# Autodesk Inventor assembly: inner
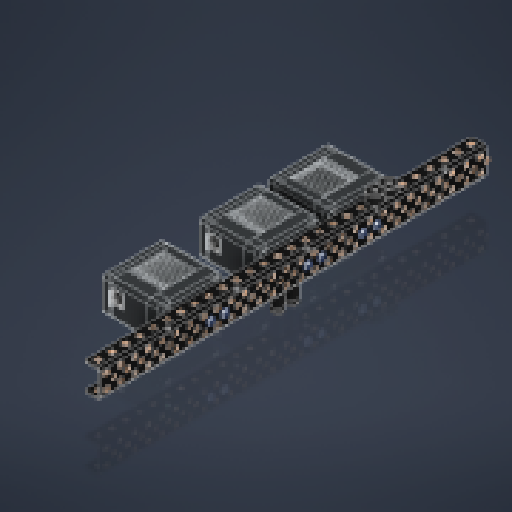
[picture p0: Inventor's stored thumbnail of the model, 512x512]
Saved by Autodesk Inventor 2024 (Build 280153000, 153)
## iProperties
Created: 2024-02-11
Part Number: inner
Document SubType Name: Assembly
Designer: Averey Ku
Author: Averey Ku
## Documents named in this file (15)
- D:\vex_robotics\hardware\cad\vroomba_v0.1\chassis\drivebay\inner.iam
- D:\vex_robotics\hardware\cad\VEX-CAD-Inventor-1.41\Structure\C Channel\Aluminum 1x2x1\Alu C 1x2x1x28.ipt
- D:\vex_robotics\hardware\cad\VEX-CAD-Inventor-1.41\Electronics\Motors with Screws\SteelM-StarS.iam
- D:\vex_robotics\hardware\cad\VEX-CAD-Inventor-1.41\Electronics\Motors with Screws.iam
- D:\vex_robotics\hardware\cad\VEX-CAD-Inventor-1.41\Motion\Shaft LS\Bearing Flat Low Profile.ipt
- D:\vex_robotics\hardware\cad\VEX-CAD-Inventor-1.41\Motion\Spacers\Spacer Nylon .500 OD\NSpacer Black .500 OD x .250.ipt
- D:\vex_robotics\hardware\cad\VEX-CAD-Inventor-1.41\Motion\Spacers\Spacer Nylon .500 OD.ipt
- D:\vex_robotics\hardware\cad\VEX-CAD-Inventor-1.41\Motion\Spacers\Washer Delrin\DWasher .500 OD x .062500.ipt
- D:\vex_robotics\hardware\cad\VEX-CAD-Inventor-1.41\Structure\Hardware\Nut Low Profile.ipt
- D:\vex_robotics\hardware\cad\VEX-CAD-Inventor-1.41\Structure\1-Post Standoff Retainer.ipt
- D:\vex_robotics\hardware\cad\VEX-CAD-Inventor-1.41\Motion\Spacers\Spacer Nylon .375 OD\NSpacer .375 OD x .500.ipt
- D:\vex_robotics\hardware\cad\VEX-CAD-Inventor-1.41\Motion\Spacers\Spacer Nylon .375 OD.ipt
- D:\vex_robotics\hardware\cad\VEX-CAD-Inventor-1.41\Motion\Spacers\Spacer Nylon .375 OD\NSpacer .375 OD x .125.ipt
- D:\vex_robotics\hardware\cad\VEX-CAD-Inventor-1.41\Motion\Spacers\Washer Steel\SWasher .375 OD x .062500.ipt
- D:\vex_robotics\hardware\cad\VEX-CAD-Inventor-1.41\Motion\Spacers\Washer Steel.ipt
## Components (22 placed, 10 different names)
1. Alu C 1x2x1x28:1 — Insert:1, Mate:1, Insert:2, Mate:2, Insert:3, Mate:3, Insert:4, Mate:4, Insert:5, Mate:5, Insert:6, Mate:6, Insert:7, Mate:7, Insert:10, Insert:11, Insert:14, Insert:15, Mate:8, Mate:9, Insert:20, Insert:21
2. SteelM-StarS:1 [sub-assembly] — Insert:3, Mate:3
3. SteelM-StarS:2 [sub-assembly] — Insert:2, Mate:2
4. SteelM-StarS:3 [sub-assembly] — Insert:1, Mate:1
5. Bearing Flat Low Profile:1 — Insert:4, Mate:4
6. Bearing Flat Low Profile:2 — Insert:5, Mate:5
7. Bearing Flat Low Profile:3 — Insert:6, Mate:6
8. Bearing Flat Low Profile:4 — Insert:7, Mate:7
9. NSpacer Black .500 OD x .250:1 — Insert:11
10. DWasher .500 OD x .062500:1
11. NSpacer Black .500 OD x .250:2 — Insert:10
12. DWasher .500 OD x .062500:2
13. Nut Low Profile:1
14. 1-Post Standoff Retainer:1 — Insert:15, Mate:8
15. Nut Low Profile:2
16. 1-Post Standoff Retainer:2 — Insert:14, Mate:9
17. NSpacer .375 OD x .500:1 — Insert:20
18. NSpacer .375 OD x .125:2
19. SWasher .375 OD x .062500:1
20. NSpacer .375 OD x .500:3 — Insert:21
21. NSpacer .375 OD x .125:4
22. SWasher .375 OD x .062500:2
## Relationships (30: Insert 21, Mate 9)
- Insert:1: Alu C 1x2x1x28:1 ↔ SteelM-StarS:3
- Mate:1: Alu C 1x2x1x28:1 ↔ SteelM-StarS:3
- Insert:2: Alu C 1x2x1x28:1 ↔ SteelM-StarS:2
- Mate:2: Alu C 1x2x1x28:1 ↔ SteelM-StarS:2
- Insert:3: Alu C 1x2x1x28:1 ↔ SteelM-StarS:1
- Mate:3: Alu C 1x2x1x28:1 ↔ SteelM-StarS:1
- Insert:4: Alu C 1x2x1x28:1 ↔ Bearing Flat Low Profile:1
- Mate:4: Alu C 1x2x1x28:1 ↔ Bearing Flat Low Profile:1
- Insert:5: Alu C 1x2x1x28:1 ↔ Bearing Flat Low Profile:2
- Mate:5: Alu C 1x2x1x28:1 ↔ Bearing Flat Low Profile:2
- Insert:6: Alu C 1x2x1x28:1 ↔ Bearing Flat Low Profile:3
- Mate:6: Alu C 1x2x1x28:1 ↔ Bearing Flat Low Profile:3
- Insert:7: Alu C 1x2x1x28:1 ↔ Bearing Flat Low Profile:4
- Mate:7: Alu C 1x2x1x28:1 ↔ Bearing Flat Low Profile:4
- [Insert]: NSpacer Black .500 OD x .250:1 ↔ DWasher .500 OD x .062500:1
- [Insert]: NSpacer Black .500 OD x .250:2 ↔ DWasher .500 OD x .062500:2
- Insert:10: Alu C 1x2x1x28:1 ↔ NSpacer Black .500 OD x .250:2
- Insert:11: Alu C 1x2x1x28:1 ↔ NSpacer Black .500 OD x .250:1
- [Insert]: Nut Low Profile:1 ↔ 1-Post Standoff Retainer:1
- [Insert]: Nut Low Profile:2 ↔ 1-Post Standoff Retainer:2
- Insert:14: Alu C 1x2x1x28:1 ↔ 1-Post Standoff Retainer:2
- Insert:15: Alu C 1x2x1x28:1 ↔ 1-Post Standoff Retainer:1
- Mate:8: Alu C 1x2x1x28:1 ↔ 1-Post Standoff Retainer:1
- Mate:9: Alu C 1x2x1x28:1 ↔ 1-Post Standoff Retainer:2
- [Insert]: NSpacer .375 OD x .125:2 ↔ SWasher .375 OD x .062500:1
- [Insert]: NSpacer .375 OD x .500:1 ↔ NSpacer .375 OD x .125:2
- [Insert]: NSpacer .375 OD x .125:4 ↔ SWasher .375 OD x .062500:2
- [Insert]: NSpacer .375 OD x .500:3 ↔ NSpacer .375 OD x .125:4
- Insert:20: Alu C 1x2x1x28:1 ↔ NSpacer .375 OD x .500:1
- Insert:21: Alu C 1x2x1x28:1 ↔ NSpacer .375 OD x .500:3
## Named parameters: d15_d39 = 0 mm, d19_d33 = 0 mm, d58_d55 = 0 mm, d59_d56 = 0 mm, d26_d58_d55 = 0 mm, d27_d59_d56 = 0 mm
